# Autodesk Inventor assembly: x_iddler
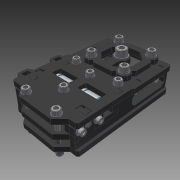
[picture p0: Inventor's stored thumbnail of the model, 180x180]
Saved by Autodesk Inventor 2014 (Build 180170000, 170)
## iProperties
Created: 2014-01-10
Part Number: x_iddler
Document SubType Name: Assembly
Designer: buben
Author: buben
## Documents named in this file (29)
- C:\Users\buben\Documents\GitHub\bacon\inventor files\assemblies\x_iddler.iam
- C:\Users\buben\Documents\GitHub\bacon\inventor files\printer parts\x_iddler_bottom.ipt
- C:\Users\buben\Documents\GitHub\bacon\inventor files\printer parts\x_iddler_wall_lower.ipt
- C:\Users\buben\Documents\GitHub\bacon\inventor files\printer parts\x_iddler_wall_upper.ipt
- C:\Users\buben\Documents\GitHub\bacon\inventor files\printer parts\x_iddler_upper_nut_stop.ipt
- C:\Users\buben\Documents\GitHub\bacon\inventor files\printer parts\x_iddler_belt_bearing_mount.ipt
- C:\Users\buben\Documents\GitHub\bacon\inventor files\printer parts\x_motor_smooth_rod_spacer.ipt
- C:\Users\buben\Documents\GitHub\bacon\inventor files\printer parts\x_motor_middle.ipt
- C:\Users\buben\Documents\GitHub\bacon\inventor files\3rd party components\linear_bearing_8\Imported Components\LU8MM\LU8MM.iam
- C:\Users\buben\Documents\GitHub\bacon\inventor files\printer parts\x_motor_top.ipt
- C:\Users\buben\Documents\GitHub\bacon\inventor files\printer parts\x_motor_lower_nut_stop.ipt
- C:\Users\buben\Documents\GitHub\bacon\inventor files\printer parts\x_iddler_c_mount.ipt
- C:\Users\buben\Documents\GitHub\bacon\inventor files\utils\washer_m5.ipt
- C:\Users\buben\Documents\Inventor\Content Center Files\R2014\en-US\ISO 4762(2)\ISO 4762 - M5 x 45ISO.ipt
- C:\Users\buben\Documents\Inventor\Content Center Files\R2014\en-US\ISO 7040\ISO 7040 - M5.ipt
- C:\Users\buben\Documents\GitHub\bacon\inventor files\utils\washer_m6.ipt
- C:\Users\buben\Documents\Inventor\Content Center Files\R2014\en-US\ISO 4762(2)\ISO 4762 - M6 x 60ISO.ipt
- C:\Users\buben\Documents\Inventor\Content Center Files\R2014\en-US\ISO 7040\ISO 7040 - M6.ipt
- C:\Users\buben\Documents\GitHub\bacon\inventor files\utils\washer_m8.ipt
- C:\Users\buben\Documents\Inventor\Content Center Files\R2014\en-US\ISO 4762(2)\ISO 4762 - M8 x 60ISO.ipt
- C:\Users\buben\Documents\Inventor\Content Center Files\R2014\en-US\ISO 7040\ISO 7040 - M8.ipt
- C:\Users\buben\Documents\GitHub\bacon\inventor files\utils\washer_m4.ipt
- C:\Users\buben\Documents\Inventor\Content Center Files\R2014\en-US\ISO 4762(2)\ISO 4762 - M4 x 20ISO.ipt
- C:\Users\buben\Documents\Inventor\Content Center Files\R2014\en-US\CSN EN 24032\ISO 4032 - M5CSN EN.ipt
- C:\Users\buben\Documents\Inventor\Content Center Files\R2014\en-US\ISO 7040\ISO 7040 - M4.ipt
- C:\Users\buben\Documents\GitHub\bacon\inventor files\3rd party components\bearing_608\Imported Components\608RS\608RS.ipt
- C:\Users\buben\Documents\GitHub\bacon\inventor files\utils\belt_guide.ipt
- C:\Users\buben\Documents\GitHub\bacon\inventor files\utils\bearing_spacer_1.ipt
- C:\Users\buben\Documents\GitHub\bacon\inventor files\utils\bearing_spacer_2.ipt
## Components (75 placed, 28 different names)
1. x_iddler_bottom:1 — Mate:1, Flush:1, Flush:2, Mate:2, Mate:3, Mate:4, Mate:5, Mate:6, Mate:7, Mate:9, Mate:10, Mate:11, Mate:12, Mate:13, Mate:14, Mate:15, Mate:16, Mate:17, Mate:18, Mate:19, Mate:53, Mate:54, Mate:55, Mate:56, Mate:57, Mate:58
2. x_iddler_wall_lower:1 — Mate:5, Mate:6, Mate:7, Mate:34, Flush:3, Mate:111, Mate:112, Mate:115, Mate:116, Mate:126, Mate:127
3. x_iddler_wall_upper:1 — Mate:2, Mate:3, Mate:4, Mate:8, Mate:20, Mate:21, Mate:22, Mate:31, Mate:32, Mate:35, Mate:37, Mate:123, Mate:124
4. x_iddler_upper_nut_stop:1 — Mate:8, Mate:9, Mate:10, Mate:36, Mate:125
5. x_iddler_belt_bearing_mount:1 — Mate:11, Mate:12, Mate:13, Mate:85, Mate:87, Mate:89, Mate:91, Mate:103, Mate:104, Mate:150
6. x_iddler_belt_bearing_mount:2 — Mate:38, Mate:39, Mate:40, Mate:77, Mate:78, Mate:79, Mate:80, Mate:81, Mate:82, Mate:83, Mate:84, Mate:101, Mate:102
7. x_motor_smooth_rod_spacer:1 — Mate:14, Mate:15, Mate:16
8. x_motor_smooth_rod_spacer:2 — Mate:17, Mate:18, Mate:19
9. x_motor_middle:1 — Mate:20, Mate:21, Mate:22, Mate:23, Mate:24, Mate:25, Mate:26, Mate:27, Mate:28, Mate:33
10. LU8MM:1 [sub-assembly] — Mate:25, Mate:26, Mate:28
11. LU8MM:2 [sub-assembly] — Mate:23, Mate:24, Mate:27, Mate:29, Mate:30
12. x_motor_top:1 — Mate:29, Mate:30, Mate:31, Mate:32, Mate:41, Mate:42, Mate:43, Mate:44, Mate:45, Mate:46, Mate:47, Mate:48, Mate:49, Mate:50, Mate:51, Mate:52
13. x_motor_lower_nut_stop:1 — Mate:33, Mate:34, Flush:3, Mate:109, Mate:110, Mate:121, Mate:128
14. x_iddler_c_mount:1 — Mate:35, Mate:36, Mate:37, Mate:38, Mate:39, Mate:40
15. CSN 02 1702 B B 5,3:1 — Mate:45, Mate:52, Insert:6
16. CSN 02 1702 B B 5,3:2 — Mate:44, Mate:50, Insert:4
17. CSN 02 1702 B B 5,3:3 — Mate:43, Mate:49, Insert:3
18. CSN 02 1702 B B 5,3:4 — Mate:41, Mate:47, Insert:1
19. CSN 02 1702 B B 5,3:5 — Mate:42, Mate:48, Insert:5
20. CSN 02 1702 B B 5,3:6 — Mate:46, Mate:51, Insert:2
21. CSN 02 1702 B B 5,3:7 — Mate:55, Mate:60, Mate:69
22. CSN 02 1702 B B 5,3:8 — Mate:58, Mate:63, Mate:65
23. CSN 02 1702 B B 5,3:9 — Mate:56, Mate:62, Mate:67
24. CSN 02 1702 B B 5,3:10 — Mate:54, Mate:61, Mate:73
25. CSN 02 1702 B B 5,3:11 — Mate:53, Mate:59, Mate:71
26. CSN 02 1702 B B 5,3:12 — Mate:57, Mate:64, Mate:75
27. ISO 4762 M5 x 45:1 — Insert:1, Mate:61, Mate:74
28. ISO 4762 M5 x 45:2 — Insert:2, Mate:60, Mate:70
29. ISO 4762 M5 x 45:3 — Insert:3, Mate:59, Mate:72
30. ISO 4762 M5 x 45:4 — Insert:4, Mate:63, Mate:66
31. ISO 4762 M5 x 45:5 — Insert:5, Mate:64, Mate:76
32. ISO 4762 M5 x 45:6 — Insert:6, Mate:62, Mate:68
33. DIN EN ISO 7040 M5:1 — Mate:67, Mate:68
34. DIN EN ISO 7040 M5:2 — Mate:65, Mate:66
35. DIN EN ISO 7040 M5:3 — Mate:69, Mate:70
36. DIN EN ISO 7040 M5:4 — Mate:71, Mate:72
37. DIN EN ISO 7040 M5:5 — Mate:73, Mate:74
38. DIN EN ISO 7040 M5:6 — Mate:75, Mate:76
39. CSN 02 1702 B B 6,4:1 — Mate:78, Mate:83, Insert:8
40. CSN 02 1702 B B 6,4:2 — Mate:79, Mate:81, Insert:9
41. CSN 02 1702 B B 6,4:3 — Mate:80, Mate:84, Insert:7
42. CSN 02 1702 B B 6,4:4 — Mate:77, Mate:82, Insert:10
43. CSN 02 1702 B B 6,4:5 — Mate:89, Mate:90, Mate:97
44. CSN 02 1702 B B 6,4:6 — Mate:85, Mate:86, Mate:93
45. CSN 02 1702 B B 6,4:7 — Mate:87, Mate:88, Mate:95
46. CSN 02 1702 B B 6,4:8 — Mate:91, Mate:92, Mate:99
47. ISO 4762 M6 x 60:4 — Insert:7, Mate:90, Mate:98
48. ISO 4762 M6 x 60:1 — Insert:8, Mate:88, Mate:96
49. ISO 4762 M6 x 60:3 — Insert:9, Mate:92, Mate:100
50. ISO 4762 M6 x 60:2 — Insert:10, Mate:86, Mate:94
51. DIN EN ISO 7040 M6:1 — Mate:93, Mate:94
52. DIN EN ISO 7040 M6:2 — Mate:95, Mate:96
53. DIN EN ISO 7040 M6:3 — Mate:97, Mate:98
54. DIN EN ISO 7040 M6:4 — Mate:99, Mate:100
55. CSN 02 1702 B B 8,4:1 — Mate:103, Mate:104, Mate:105
56. CSN 02 1702 B B 8,4:2 — Mate:101, Mate:102, Insert:11
57. ISO 4762 M8 x 60:1 — Insert:11, Mate:106, Mate:151
58. DIN EN ISO 7040 M8:1 — Mate:105, Mate:106
59. CSN 02 1702 B B 4,3:1 — Mate:111, Mate:115, Insert:14
60. CSN 02 1702 B B 4,3:2 — Mate:112, Mate:116, Insert:15
61. CSN 02 1702 B B 4,3:7 — Mate:109, Mate:122, Mate:129
62. CSN 02 1702 B B 4,3:8 — Mate:110, Mate:121, Mate:131
63. ISO 4762 M4 x 20:3 — Insert:14, Mate:122, Mate:130
64. ISO 4762 M4 x 20:4 — Insert:15, Mate:132
65. CSN EN 24032 M5:1 — Mate:123, Mate:124, Mate:125
66. CSN EN 24032 M5:2 — Mate:126, Mate:127, Mate:128
67. DIN EN ISO 7040 M4:3 — Mate:131, Mate:132
68. DIN EN ISO 7040 M4:4 — Mate:129, Mate:130
69. 608RS:1 — Mate:137, Mate:138, Mate:141, Mate:142, Mate:143, Mate:146, Mate:147
70. belt_guide:1 — Mate:137, Mate:138, Mate:139, Mate:140
71. belt_guide:2 — Mate:139, Mate:140, Mate:141
72. CSN 02 1702 B B 8,4:3 — Mate:144, Mate:145, Mate:150, Mate:151
73. CSN 02 1702 B B 8,4:4 — Mate:148, Mate:149
74. bearing_spacer_1:1 — Mate:142, Mate:143, Mate:144, Mate:145
75. bearing_spacer_2:1 — Mate:146, Mate:147, Mate:148, Mate:149
## Relationships (155: Mate 139, Insert 13, Flush 3)
- Mate:1: x_iddler_bottom:1
- Flush:1: x_iddler_bottom:1
- Flush:2: x_iddler_bottom:1
- Mate:2: x_iddler_bottom:1 ↔ x_iddler_wall_upper:1
- Mate:3: x_iddler_bottom:1 ↔ x_iddler_wall_upper:1
- Mate:4: x_iddler_bottom:1 ↔ x_iddler_wall_upper:1
- Mate:5: x_iddler_bottom:1 ↔ x_iddler_wall_lower:1
- Mate:6: x_iddler_bottom:1 ↔ x_iddler_wall_lower:1
- Mate:7: x_iddler_bottom:1 ↔ x_iddler_wall_lower:1
- Mate:8: x_iddler_wall_upper:1 ↔ x_iddler_upper_nut_stop:1
- Mate:9: x_iddler_bottom:1 ↔ x_iddler_upper_nut_stop:1
- Mate:10: x_iddler_bottom:1 ↔ x_iddler_upper_nut_stop:1
- Mate:11: x_iddler_bottom:1 ↔ x_iddler_belt_bearing_mount:1
- Mate:12: x_iddler_bottom:1 ↔ x_iddler_belt_bearing_mount:1
- Mate:13: x_iddler_bottom:1 ↔ x_iddler_belt_bearing_mount:1
- Mate:14: x_iddler_bottom:1 ↔ x_motor_smooth_rod_spacer:1
- Mate:15: x_iddler_bottom:1 ↔ x_motor_smooth_rod_spacer:1
- Mate:16: x_iddler_bottom:1 ↔ x_motor_smooth_rod_spacer:1
- Mate:17: x_iddler_bottom:1 ↔ x_motor_smooth_rod_spacer:2
- Mate:18: x_iddler_bottom:1 ↔ x_motor_smooth_rod_spacer:2
- Mate:19: x_iddler_bottom:1 ↔ x_motor_smooth_rod_spacer:2
- Mate:20: x_iddler_wall_upper:1 ↔ x_motor_middle:1
- Mate:21: x_iddler_wall_upper:1 ↔ x_motor_middle:1
- Mate:22: x_iddler_wall_upper:1 ↔ x_motor_middle:1
- Mate:23 (7.5 mm): x_motor_middle:1 ↔ LU8MM:2
- Mate:24 (7.5 mm): x_motor_middle:1 ↔ LU8MM:2
- Mate:25 (7.5 mm): x_motor_middle:1 ↔ LU8MM:1
- Mate:26 (7.5 mm): x_motor_middle:1 ↔ LU8MM:1
- Mate:27 (0.5 mm): x_motor_middle:1 ↔ LU8MM:2
- Mate:28 (0.5 mm): x_motor_middle:1 ↔ LU8MM:1
- Mate:29 (7.5 mm): LU8MM:2 ↔ x_motor_top:1
- Mate:30 (7.5 mm): LU8MM:2 ↔ x_motor_top:1
- Mate:31: x_iddler_wall_upper:1 ↔ x_motor_top:1
- Mate:32: x_iddler_wall_upper:1 ↔ x_motor_top:1
- Mate:33: x_motor_middle:1 ↔ x_motor_lower_nut_stop:1
- Mate:34: x_iddler_wall_lower:1 ↔ x_motor_lower_nut_stop:1
- Flush:3: x_iddler_wall_lower:1 ↔ x_motor_lower_nut_stop:1
- Mate:35: x_iddler_wall_upper:1 ↔ x_iddler_c_mount:1
- Mate:36: x_iddler_upper_nut_stop:1 ↔ x_iddler_c_mount:1
- Mate:37: x_iddler_wall_upper:1 ↔ x_iddler_c_mount:1
- Mate:38: x_iddler_belt_bearing_mount:2 ↔ x_iddler_c_mount:1
- Mate:39: x_iddler_belt_bearing_mount:2 ↔ x_iddler_c_mount:1
- Mate:40: x_iddler_belt_bearing_mount:2 ↔ x_iddler_c_mount:1
- Mate:41: x_motor_top:1 ↔ CSN 02 1702 B B 5,3:4
- Mate:42: x_motor_top:1 ↔ CSN 02 1702 B B 5,3:5
- Mate:43: x_motor_top:1 ↔ CSN 02 1702 B B 5,3:3
- Mate:44: x_motor_top:1 ↔ CSN 02 1702 B B 5,3:2
- Mate:45: x_motor_top:1 ↔ CSN 02 1702 B B 5,3:1
- Mate:46: x_motor_top:1 ↔ CSN 02 1702 B B 5,3:6
- Mate:47: x_motor_top:1 ↔ CSN 02 1702 B B 5,3:4
- Mate:48: x_motor_top:1 ↔ CSN 02 1702 B B 5,3:5
- Mate:49: x_motor_top:1 ↔ CSN 02 1702 B B 5,3:3
- Mate:50: x_motor_top:1 ↔ CSN 02 1702 B B 5,3:2
- Mate:51: x_motor_top:1 ↔ CSN 02 1702 B B 5,3:6
- Mate:52: x_motor_top:1 ↔ CSN 02 1702 B B 5,3:1
- Insert:1: CSN 02 1702 B B 5,3:4 ↔ ISO 4762 M5 x 45:1
- Insert:2: CSN 02 1702 B B 5,3:6 ↔ ISO 4762 M5 x 45:2
- Insert:3: CSN 02 1702 B B 5,3:3 ↔ ISO 4762 M5 x 45:3
- Insert:4: CSN 02 1702 B B 5,3:2 ↔ ISO 4762 M5 x 45:4
- Insert:5: CSN 02 1702 B B 5,3:5 ↔ ISO 4762 M5 x 45:5
- Insert:6: CSN 02 1702 B B 5,3:1 ↔ ISO 4762 M5 x 45:6
- Mate:53: x_iddler_bottom:1 ↔ CSN 02 1702 B B 5,3:11
- Mate:54: x_iddler_bottom:1 ↔ CSN 02 1702 B B 5,3:10
- Mate:55: x_iddler_bottom:1 ↔ CSN 02 1702 B B 5,3:7
- Mate:56: x_iddler_bottom:1 ↔ CSN 02 1702 B B 5,3:9
- Mate:57: x_iddler_bottom:1 ↔ CSN 02 1702 B B 5,3:12
- Mate:58: x_iddler_bottom:1 ↔ CSN 02 1702 B B 5,3:8
- Mate:59: CSN 02 1702 B B 5,3:11 ↔ ISO 4762 M5 x 45:3
- Mate:60: CSN 02 1702 B B 5,3:7 ↔ ISO 4762 M5 x 45:2
- Mate:61: CSN 02 1702 B B 5,3:10 ↔ ISO 4762 M5 x 45:1
- Mate:62: CSN 02 1702 B B 5,3:9 ↔ ISO 4762 M5 x 45:6
- Mate:63: CSN 02 1702 B B 5,3:8 ↔ ISO 4762 M5 x 45:4
- Mate:64: CSN 02 1702 B B 5,3:12 ↔ ISO 4762 M5 x 45:5
- Mate:65: CSN 02 1702 B B 5,3:8 ↔ DIN EN ISO 7040 M5:2
- Mate:66: ISO 4762 M5 x 45:4 ↔ DIN EN ISO 7040 M5:2
- Mate:67: CSN 02 1702 B B 5,3:9 ↔ DIN EN ISO 7040 M5:1
- Mate:68: ISO 4762 M5 x 45:6 ↔ DIN EN ISO 7040 M5:1
- Mate:69: CSN 02 1702 B B 5,3:7 ↔ DIN EN ISO 7040 M5:3
- Mate:70: ISO 4762 M5 x 45:2 ↔ DIN EN ISO 7040 M5:3
- Mate:71: CSN 02 1702 B B 5,3:11 ↔ DIN EN ISO 7040 M5:4
- Mate:72: ISO 4762 M5 x 45:3 ↔ DIN EN ISO 7040 M5:4
- Mate:73: CSN 02 1702 B B 5,3:10 ↔ DIN EN ISO 7040 M5:5
- Mate:74: ISO 4762 M5 x 45:1 ↔ DIN EN ISO 7040 M5:5
- Mate:75: CSN 02 1702 B B 5,3:12 ↔ DIN EN ISO 7040 M5:6
- Mate:76: ISO 4762 M5 x 45:5 ↔ DIN EN ISO 7040 M5:6
- Mate:77: x_iddler_belt_bearing_mount:2 ↔ CSN 02 1702 B B 6,4:4
- Mate:78: x_iddler_belt_bearing_mount:2 ↔ CSN 02 1702 B B 6,4:1
- Mate:79: x_iddler_belt_bearing_mount:2 ↔ CSN 02 1702 B B 6,4:2
- Mate:80: x_iddler_belt_bearing_mount:2 ↔ CSN 02 1702 B B 6,4:3
- Mate:81: x_iddler_belt_bearing_mount:2 ↔ CSN 02 1702 B B 6,4:2
- Mate:82: x_iddler_belt_bearing_mount:2 ↔ CSN 02 1702 B B 6,4:4
- Mate:83: x_iddler_belt_bearing_mount:2 ↔ CSN 02 1702 B B 6,4:1
- Mate:84: x_iddler_belt_bearing_mount:2 ↔ CSN 02 1702 B B 6,4:3
- Insert:7: CSN 02 1702 B B 6,4:3 ↔ ISO 4762 M6 x 60:4
- Insert:8: CSN 02 1702 B B 6,4:1 ↔ ISO 4762 M6 x 60:1
- Insert:9: CSN 02 1702 B B 6,4:2 ↔ ISO 4762 M6 x 60:3
- Insert:10: CSN 02 1702 B B 6,4:4 ↔ ISO 4762 M6 x 60:2
- Mate:85: x_iddler_belt_bearing_mount:1 ↔ CSN 02 1702 B B 6,4:6
- Mate:86: CSN 02 1702 B B 6,4:6 ↔ ISO 4762 M6 x 60:2
- Mate:87: x_iddler_belt_bearing_mount:1 ↔ CSN 02 1702 B B 6,4:7
- Mate:88: CSN 02 1702 B B 6,4:7 ↔ ISO 4762 M6 x 60:1
- Mate:89: x_iddler_belt_bearing_mount:1 ↔ CSN 02 1702 B B 6,4:5
- Mate:90: CSN 02 1702 B B 6,4:5 ↔ ISO 4762 M6 x 60:4
- Mate:91: x_iddler_belt_bearing_mount:1 ↔ CSN 02 1702 B B 6,4:8
- Mate:92: CSN 02 1702 B B 6,4:8 ↔ ISO 4762 M6 x 60:3
- Mate:93: CSN 02 1702 B B 6,4:6 ↔ DIN EN ISO 7040 M6:1
- Mate:94: ISO 4762 M6 x 60:2 ↔ DIN EN ISO 7040 M6:1
- Mate:95: CSN 02 1702 B B 6,4:7 ↔ DIN EN ISO 7040 M6:2
- Mate:96: ISO 4762 M6 x 60:1 ↔ DIN EN ISO 7040 M6:2
- Mate:97: CSN 02 1702 B B 6,4:5 ↔ DIN EN ISO 7040 M6:3
- Mate:98: ISO 4762 M6 x 60:4 ↔ DIN EN ISO 7040 M6:3
- Mate:99: CSN 02 1702 B B 6,4:8 ↔ DIN EN ISO 7040 M6:4
- Mate:100: ISO 4762 M6 x 60:3 ↔ DIN EN ISO 7040 M6:4
- Mate:101: x_iddler_belt_bearing_mount:2 ↔ CSN 02 1702 B B 8,4:2
- Mate:102: x_iddler_belt_bearing_mount:2 ↔ CSN 02 1702 B B 8,4:2
- Mate:103: x_iddler_belt_bearing_mount:1 ↔ CSN 02 1702 B B 8,4:1
- Mate:104: x_iddler_belt_bearing_mount:1 ↔ CSN 02 1702 B B 8,4:1
- Insert:11: CSN 02 1702 B B 8,4:2 ↔ ISO 4762 M8 x 60:1
- Mate:105: CSN 02 1702 B B 8,4:1 ↔ DIN EN ISO 7040 M8:1
- Mate:106: ISO 4762 M8 x 60:1 ↔ DIN EN ISO 7040 M8:1
- Mate:109: x_motor_lower_nut_stop:1 ↔ CSN 02 1702 B B 4,3:7
- Mate:110: x_motor_lower_nut_stop:1 ↔ CSN 02 1702 B B 4,3:8
- Mate:111: x_iddler_wall_lower:1 ↔ CSN 02 1702 B B 4,3:1
- Mate:112: x_iddler_wall_lower:1 ↔ CSN 02 1702 B B 4,3:2
- Mate:115: x_iddler_wall_lower:1 ↔ CSN 02 1702 B B 4,3:1
- Mate:116: x_iddler_wall_lower:1 ↔ CSN 02 1702 B B 4,3:2
- Insert:14: CSN 02 1702 B B 4,3:1 ↔ ISO 4762 M4 x 20:3
- Insert:15: CSN 02 1702 B B 4,3:2 ↔ ISO 4762 M4 x 20:4
- Mate:121: x_motor_lower_nut_stop:1 ↔ CSN 02 1702 B B 4,3:8
- Mate:122: CSN 02 1702 B B 4,3:7 ↔ ISO 4762 M4 x 20:3
- Mate:123: x_iddler_wall_upper:1 ↔ CSN EN 24032 M5:1
- Mate:124: x_iddler_wall_upper:1 ↔ CSN EN 24032 M5:1
- Mate:125: x_iddler_upper_nut_stop:1 ↔ CSN EN 24032 M5:1
- Mate:126: x_iddler_wall_lower:1 ↔ CSN EN 24032 M5:2
- Mate:127: x_iddler_wall_lower:1 ↔ CSN EN 24032 M5:2
- Mate:128: x_motor_lower_nut_stop:1 ↔ CSN EN 24032 M5:2
- Mate:129: CSN 02 1702 B B 4,3:7 ↔ DIN EN ISO 7040 M4:4
- Mate:130: ISO 4762 M4 x 20:3 ↔ DIN EN ISO 7040 M4:4
- Mate:131: CSN 02 1702 B B 4,3:8 ↔ DIN EN ISO 7040 M4:3
- Mate:132: ISO 4762 M4 x 20:4 ↔ DIN EN ISO 7040 M4:3
- Mate:137: 608RS:1 ↔ belt_guide:1
- Mate:138: 608RS:1 ↔ belt_guide:1
- Mate:139: belt_guide:1 ↔ belt_guide:2
- Mate:140: belt_guide:1 ↔ belt_guide:2
- Mate:141: 608RS:1 ↔ belt_guide:2
- Mate:142: 608RS:1 ↔ bearing_spacer_1:1
- Mate:143: 608RS:1 ↔ bearing_spacer_1:1
- Mate:144: CSN 02 1702 B B 8,4:3 ↔ bearing_spacer_1:1
- Mate:145: CSN 02 1702 B B 8,4:3 ↔ bearing_spacer_1:1
- Mate:146: 608RS:1 ↔ bearing_spacer_2:1
- Mate:147: 608RS:1 ↔ bearing_spacer_2:1
- Mate:148: CSN 02 1702 B B 8,4:4 ↔ bearing_spacer_2:1
- Mate:149: CSN 02 1702 B B 8,4:4 ↔ bearing_spacer_2:1
- Mate:150: x_iddler_belt_bearing_mount:1 ↔ CSN 02 1702 B B 8,4:3
- Mate:151: ISO 4762 M8 x 60:1 ↔ CSN 02 1702 B B 8,4:3
